# Autodesk Inventor assembly: Сборка_редуктор+муфта
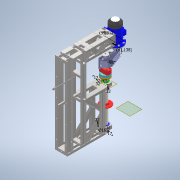
[picture p0: Inventor's stored thumbnail of the model, 180x180]
Saved by Autodesk Inventor 2021 (Build 250183000, 183)
## iProperties
Created: 2023-04-27
Part Number: Сборка_редуктор+муфта
Document SubType Name: Assembly
Designer: gdevc
Mass: 171768 g
Surface Area: 70066.4 cm^2
Volume: 31927.6 cm^3
Density: 5.37994 g/cm^3
Author: gdevc
## Documents named in this file (14)
- C:\Users\gdevc\OneDrive\Рабочий стол\Курсач\DetaliMashine\Новая папка\Сборка_редуктора+муфта\Сборка_редуктор+муфта.iam
- C:\Users\gdevc\OneDrive\Рабочий стол\Курсач\DetaliMashine\Новая папка\Сборка_новая.iam
- C:\Users\gdevc\OneDrive\Рабочий стол\Курсач\DetaliMashine\Новая папка\Муфта в сборе.iam
- C:\Users\gdevc\OneDrive\Рабочий стол\Курсач\DetaliMashine\Новая папка\Приводной валл\Сборка вала.iam
- C:\Users\gdevc\OneDrive\Рабочий стол\Курсач\DetaliMashine\Новая папка\Рама\Рама_сварная_v.2.iam
- C:\Users\gdevc\OneDrive\Рабочий стол\Курсач\DetaliMashine\Новая папка\Сборка_редуктора+муфта\Фундаментальная хуйня1.ipt
- C:\Users\gdevc\OneDrive\Документы\Inventor\Content Center Files\R2021\ru-RU\Bolt GOST 7798-78\Болт M12-6g×30(S18) ГОСТ 7798-70.ipt
- C:\Users\gdevc\OneDrive\Документы\Inventor\Content Center Files\R2021\ru-RU\GOST 5915-70\Гайка M12-6H ГОСТ 5915-70(1).ipt
- C:\Users\gdevc\OneDrive\Документы\Inventor\Content Center Files\R2021\ru-RU\Bolt GOST 7798-78\Болт M16-6g×45(S24) ГОСТ 7798-70.ipt
- C:\Users\gdevc\OneDrive\Документы\Inventor\Content Center Files\R2021\ru-RU\Nut GOST ISO 8673-2014\Копия Копия гайки M16x1,5-6H ГОСТ 5915-70.ipt
- C:\Users\gdevc\OneDrive\Документы\Inventor\Content Center Files\R2021\ru-RU\Bolt GOST 7798-78\Болт M10-6g×10(S16) ГОСТ 7798-70.ipt
- C:\Users\gdevc\OneDrive\Рабочий стол\Курсач\DetaliMashine\Новая папка\Рама\Шпилька.ipt
- C:\Users\gdevc\OneDrive\Документы\Inventor\Content Center Files\R2021\ru-RU\GOST 5915-70\Гайка M16-6H ГОСТ 5915-70(1).ipt
- C:\Users\gdevc\OneDrive\Документы\Inventor\Content Center Files\R2021\ru-RU\GOST 11371-78  A\Шайба 16 ГОСТ 11371-78.ipt
## Components (44 placed, 13 different names)
1. Сборка_новая:1 [sub-assembly] — Совмещение:1, Совмещение:7, Совмещение:8, Совмещение:19, Совмещение:20, Совмещение:21, Совмещение:22, Совмещение:23, Совмещение:24, Совмещение:25, Совмещение:26, Совмещение:27, Совмещение:28, Заподлицо:3, Совмещение:30
2. Муфта в сборе:1 [sub-assembly] — Совмещение:1, Угол:1, Совмещение:3
3. Сборка вала:1 [sub-assembly] — Совмещение:3, Угол:2, Совмещение:4, Заподлицо:1, Заподлицо:2, Совмещение:11, Совмещение:13, Совмещение:32, Совмещение:35, Совмещение:40, Совмещение:44
4. Рама_сварная_v.2:1 [sub-assembly] — Угол:3, Совмещение:4, Заподлицо:1, Заподлицо:2, Совмещение:5, Совмещение:6, Совмещение:10, Совмещение:16, Совмещение:18
5. Фундаментальная хуйня1:1 — Совмещение:5, Совмещение:6
6. Болт ГОСТ 7798-70 M12-6g×30(S18):1 — Совмещение:7, Совмещение:8, Совмещение:9
7. Гайка ГОСТ 5915-70 M12:1 — Совмещение:9, Совмещение:10
8. Болт ГОСТ 7798-70 M16-6g×45(S24):1 — Совмещение:11, Совмещение:15, Совмещение:31, Совмещение:33
9. Болт ГОСТ 7798-70 M16-6g×45(S24):2 — Совмещение:13, Совмещение:17, Совмещение:34, Совмещение:36
10. Гайка ГОСТ ISO 8673-2014 M16x1,5:1 — Совмещение:15, Совмещение:16
11. Гайка ГОСТ ISO 8673-2014 M16x1,5:2 — Совмещение:17, Совмещение:18
12. Болт ГОСТ 7798-70 M10-6g×10(S16):1 — Совмещение:24
13. Болт ГОСТ 7798-70 M10-6g×10(S16):2 — Совмещение:23
14. Болт ГОСТ 7798-70 M10-6g×10(S16):3 — Совмещение:22
15. Болт ГОСТ 7798-70 M10-6g×10(S16):4 — Совмещение:19
16. Болт ГОСТ 7798-70 M10-6g×10(S16):5 — Совмещение:21
17. Болт ГОСТ 7798-70 M10-6g×10(S16):6 — Совмещение:20
18. Болт ГОСТ 7798-70 M10-6g×10(S16):7 — Совмещение:26
19. Болт ГОСТ 7798-70 M10-6g×10(S16):8 — Совмещение:27
20. Болт ГОСТ 7798-70 M10-6g×10(S16):9 — Совмещение:25
21. Шайба  ГОСТ 11371-78 17:1 — Совмещение:31, Совмещение:32, Совмещение:33
22. Шайба  ГОСТ 11371-78 17:2 — Совмещение:34, Совмещение:35, Совмещение:36
23. Болт ГОСТ 7798-70 M16-6g×45(S24):3 — Совмещение:37, Совмещение:38, Совмещение:39, Совмещение:40
24. Гайка ГОСТ ISO 8673-2014 M16x1,5:3 — Совмещение:37
25. Шайба  ГОСТ 11371-78 17:3 — Совмещение:38, Совмещение:39
26. Болт ГОСТ 7798-70 M16-6g×45(S24):4 — Совмещение:41, Совмещение:42, Совмещение:43, Совмещение:44
27. Гайка ГОСТ ISO 8673-2014 M16x1,5:4 — Совмещение:41
28. Шайба  ГОСТ 11371-78 17:4 — Совмещение:42, Совмещение:43
29. Шпилька:1 — Совмещение:28, Заподлицо:3, Совмещение:29
30. Гайка ГОСТ 5915-70 M16:1 — Совмещение:29, Совмещение:30
31. Шпилька:2
32. Гайка ГОСТ 5915-70 M16:2
33. Шпилька:3
34. Гайка ГОСТ 5915-70 M16:3
35. Шпилька:4
36. Гайка ГОСТ 5915-70 M16:4
37. Шпилька:5
38. Гайка ГОСТ 5915-70 M16:5
39. Шпилька:6
40. Гайка ГОСТ 5915-70 M16:6
41. Шпилька:7
42. Гайка ГОСТ 5915-70 M16:7
43. Шпилька:8
44. Гайка ГОСТ 5915-70 M16:8
## Component patterns: (8 elements, first: Шпилька:1 + Гайка ГОСТ 5915-70 M16:1)
## Relationships (47: Mate 41, Angle 3, Flush 3)
- Совмещение:1 [Mate]: Сборка_новая:1 ↔ Муфта в сборе:1
- Угол:1 [Angle] (180 deg): Муфта в сборе:1
- Совмещение:3 [Mate]: Муфта в сборе:1 ↔ Сборка вала:1
- Угол:2 [Angle] (0 deg): Сборка вала:1
- Угол:3 [Angle] (0 deg): Рама_сварная_v.2:1
- Совмещение:4 [Mate]: Сборка вала:1 ↔ Рама_сварная_v.2:1
- Заподлицо:1 [Flush]: Сборка вала:1 ↔ Рама_сварная_v.2:1
- Заподлицо:2 [Flush]: Сборка вала:1 ↔ Рама_сварная_v.2:1
- Совмещение:5 [Mate]: Рама_сварная_v.2:1 ↔ Фундаментальная хуйня1:1
- Совмещение:6 [Mate]: Рама_сварная_v.2:1 ↔ Фундаментальная хуйня1:1
- Совмещение:7 [Mate]: Сборка_новая:1 ↔ Болт ГОСТ 7798-70 M12-6g×30(S18):1
- Совмещение:8 [Mate]: Сборка_новая:1 ↔ Болт ГОСТ 7798-70 M12-6g×30(S18):1
- Совмещение:9 [Mate]: Болт ГОСТ 7798-70 M12-6g×30(S18):1 ↔ Гайка ГОСТ 5915-70 M12:1
- Совмещение:10 [Mate]: Рама_сварная_v.2:1 ↔ Гайка ГОСТ 5915-70 M12:1
- Совмещение:11 [Mate]: Сборка вала:1 ↔ Болт ГОСТ 7798-70 M16-6g×45(S24):1
- Совмещение:13 [Mate]: Сборка вала:1 ↔ Болт ГОСТ 7798-70 M16-6g×45(S24):2
- Совмещение:15 [Mate]: Болт ГОСТ 7798-70 M16-6g×45(S24):1 ↔ Гайка ГОСТ ISO 8673-2014 M16x1,5:1
- Совмещение:16 [Mate]: Рама_сварная_v.2:1 ↔ Гайка ГОСТ ISO 8673-2014 M16x1,5:1
- Совмещение:17 [Mate]: Болт ГОСТ 7798-70 M16-6g×45(S24):2 ↔ Гайка ГОСТ ISO 8673-2014 M16x1,5:2
- Совмещение:18 [Mate]: Рама_сварная_v.2:1 ↔ Гайка ГОСТ ISO 8673-2014 M16x1,5:2
- Совмещение:19 [Mate]: Сборка_новая:1 ↔ Болт ГОСТ 7798-70 M10-6g×10(S16):4
- Совмещение:20 [Mate]: Сборка_новая:1 ↔ Болт ГОСТ 7798-70 M10-6g×10(S16):6
- Совмещение:21 [Mate]: Сборка_новая:1 ↔ Болт ГОСТ 7798-70 M10-6g×10(S16):5
- Совмещение:22 [Mate]: Сборка_новая:1 ↔ Болт ГОСТ 7798-70 M10-6g×10(S16):3
- Совмещение:23 [Mate]: Сборка_новая:1 ↔ Болт ГОСТ 7798-70 M10-6g×10(S16):2
- Совмещение:24 [Mate]: Сборка_новая:1 ↔ Болт ГОСТ 7798-70 M10-6g×10(S16):1
- Совмещение:25 [Mate]: Сборка_новая:1 ↔ Болт ГОСТ 7798-70 M10-6g×10(S16):9
- Совмещение:26 [Mate]: Сборка_новая:1 ↔ Болт ГОСТ 7798-70 M10-6g×10(S16):7
- Совмещение:27 [Mate]: Сборка_новая:1 ↔ Болт ГОСТ 7798-70 M10-6g×10(S16):8
- Совмещение:28 [Mate]: Сборка_новая:1 ↔ Шпилька:1
- Заподлицо:3 [Flush] (2 mm): Сборка_новая:1 ↔ Шпилька:1
- Совмещение:29 [Mate]: Шпилька:1 ↔ Гайка ГОСТ 5915-70 M16:1
- Совмещение:30 [Mate]: Сборка_новая:1 ↔ Гайка ГОСТ 5915-70 M16:1
- Совмещение:31 [Mate]: Болт ГОСТ 7798-70 M16-6g×45(S24):1 ↔ Шайба  ГОСТ 11371-78 17:1
- Совмещение:32 [Mate]: Сборка вала:1 ↔ Шайба  ГОСТ 11371-78 17:1
- Совмещение:33 [Mate]: Болт ГОСТ 7798-70 M16-6g×45(S24):1 ↔ Шайба  ГОСТ 11371-78 17:1
- Совмещение:34 [Mate]: Болт ГОСТ 7798-70 M16-6g×45(S24):2 ↔ Шайба  ГОСТ 11371-78 17:2
- Совмещение:35 [Mate]: Сборка вала:1 ↔ Шайба  ГОСТ 11371-78 17:2
- Совмещение:36 [Mate]: Болт ГОСТ 7798-70 M16-6g×45(S24):2 ↔ Шайба  ГОСТ 11371-78 17:2
- Совмещение:37 [Mate]: Болт ГОСТ 7798-70 M16-6g×45(S24):3 ↔ Гайка ГОСТ ISO 8673-2014 M16x1,5:3
- Совмещение:38 [Mate]: Болт ГОСТ 7798-70 M16-6g×45(S24):3 ↔ Шайба  ГОСТ 11371-78 17:3
- Совмещение:39 [Mate]: Болт ГОСТ 7798-70 M16-6g×45(S24):3 ↔ Шайба  ГОСТ 11371-78 17:3
- Совмещение:40 [Mate]: Сборка вала:1 ↔ Болт ГОСТ 7798-70 M16-6g×45(S24):3
- Совмещение:41 [Mate]: Болт ГОСТ 7798-70 M16-6g×45(S24):4 ↔ Гайка ГОСТ ISO 8673-2014 M16x1,5:4
- Совмещение:42 [Mate]: Болт ГОСТ 7798-70 M16-6g×45(S24):4 ↔ Шайба  ГОСТ 11371-78 17:4
- Совмещение:43 [Mate]: Болт ГОСТ 7798-70 M16-6g×45(S24):4 ↔ Шайба  ГОСТ 11371-78 17:4
- Совмещение:44 [Mate]: Сборка вала:1 ↔ Болт ГОСТ 7798-70 M16-6g×45(S24):4
